# Autodesk Inventor assembly: Resistencia
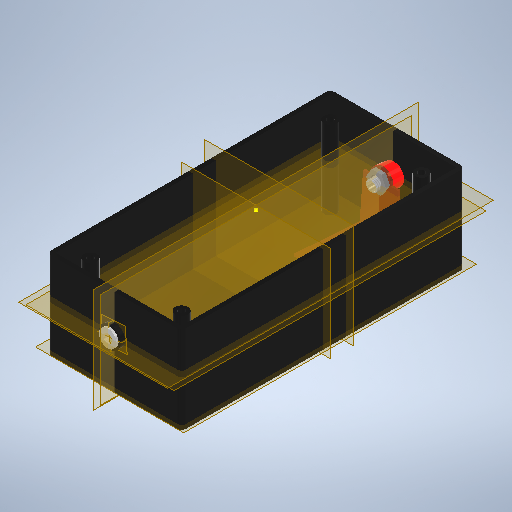
[picture p0: Inventor's stored thumbnail of the model, 512x512]
Saved by Autodesk Inventor 2026 (Build 300175050, 175E)
## iProperties
Created: 2025-05-26
Part Number: Resistencia
Document SubType Name: Assembly
Designer: alex
Author: alex
## Documents named in this file (8)
- C:\Users\alex\Desktop\Resistencia.iam
- C:\Users\alex\Desktop\Resistencia_Cuerpo.ipt
- C:\Users\alex\Desktop\Resistencia_Tornillo.ipt
- C:\Users\alex\Desktop\Resistencia_Arandela_1.ipt
- C:\Users\alex\Desktop\Resistencia_Arandela_2.ipt
- C:\Users\alex\Desktop\Resistencia_Lamina.ipt
- C:\Users\alex\Desktop\Resistencia_Tapa.ipt
- C:\Users\alex\Desktop\Resistencia_Tuerca.ipt
## Components (11 placed, 7 different names)
1. Resistencia_Cuerpo:1 — De rotación:3, De rotación:4, De rotación:5, Coincidencia:2, De rotación:7, Coincidencia:3
2. Resistencia_Tornillo:1 — De rotación:1
3. Resistencia_Arandela_1:1 — De rotación:1, De rotación:3, Coincidencia:3
4. Resistencia_Arandela_2:1 — De rotación:4, De rotación:6
5. Resistencia_Tornillo:2
6. Resistencia_Arandela_1:2 — De rotación:5
7. Resistencia_Lamina:2 — Cilíndrica:1, De rotación:8
8. Resistencia_Arandela_2:2 — Coincidencia:2, Cilíndrica:1
9. Resistencia_Lamina:3 — De rotación:6
10. Resistencia_Tapa:1 — De rotación:7
11. Resistencia_Tuerca:1 — De rotación:8
## Relationships (11: RevoluteJoint 8, Mate 2, CylindricalJoint 1)
- De rotación:1 [RevoluteJoint]: Resistencia_Tornillo:1 ↔ Resistencia_Arandela_1:1
- [RevoluteJoint]: Resistencia_Tornillo:2 ↔ Resistencia_Arandela_1:2
- De rotación:3 [RevoluteJoint]: Resistencia_Cuerpo:1 ↔ Resistencia_Arandela_1:1
- De rotación:4 [RevoluteJoint]: Resistencia_Cuerpo:1 ↔ Resistencia_Arandela_2:1
- De rotación:5 [RevoluteJoint]: Resistencia_Cuerpo:1 ↔ Resistencia_Arandela_1:2
- Coincidencia:2 [Mate]: Resistencia_Cuerpo:1 ↔ Resistencia_Arandela_2:2
- Cilíndrica:1 [CylindricalJoint]: Resistencia_Lamina:2 ↔ Resistencia_Arandela_2:2
- De rotación:6 [RevoluteJoint]: Resistencia_Arandela_2:1 ↔ Resistencia_Lamina:3
- De rotación:7 [RevoluteJoint] (3 mm): Resistencia_Cuerpo:1 ↔ Resistencia_Tapa:1
- Coincidencia:3 [Mate]: Resistencia_Cuerpo:1 ↔ Resistencia_Arandela_1:1
- De rotación:8 [RevoluteJoint]: Resistencia_Lamina:2 ↔ Resistencia_Tuerca:1
## Named parameters: d2_d0 = 0 mm, d3_d1 = 89.27414 deg
